# Autodesk Inventor assembly: LinearLift12in
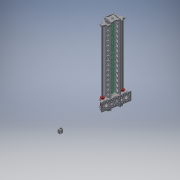
[picture p0: Inventor's stored thumbnail of the model, 180x180]
Saved by Autodesk Inventor 2018 (Build 220112000, 112)
## iProperties
Created: 2017-11-27
Part Number: LinearLift12in
Document SubType Name: Assembly
Designer: ball
Author: ball
## Documents named in this file (12)
- C:\FTC\FTC8863CAD\2017Robot\LinearLift12in.iam
- C:\FTC\FTC8863CAD\Actobotics\585 parts\585456.ipt
- C:\FTC\FTC8863CAD\Actobotics\585 parts\585634.ipt
- C:\FTC\FTC8863CAD\Actobotics\634 parts\634314.ipt
- C:\FTC\FTC8863CAD\Actobotics\535 parts\535094 assembly.ipt
- C:\FTC\FTC8863CAD\Actobotics\634 parts\634050.ipt
- C:\FTC\FTC8863CAD\Actobotics\545 parts\545314.ipt
- C:\FTC\FTC8863CAD\Actobotics\585 parts\585546.ipt
- C:\FTC\FTC8863CAD\Actobotics\535 parts\535226.ipt
- C:\FTC\FTC8863CAD\Actobotics\585 parts\585640.ipt
- C:\FTC\FTC8863CAD\Actobotics\585 parts\585722.ipt
- C:\FTC\FTC8863CAD\Actobotics\525 parts\625052 assembly.ipt
## Components (19 placed, 11 different names)
1. 585456:1 — Mate:1, Mate:2, Mate:3, Mate:7, Mate:8, Mate:9, Mate:10, Mate:14, Mate:15, Mate:16, Mate:17, Mate:38, Mate:39, Mate:40, Mate:41
2. 585634:1 — Mate:7, Mate:37, Mate:38, Mate:39
3. 585634:2 — Mate:1, Mate:2, Mate:3, Mate:4, Flush:1
4. 585634:3 — Mate:8, Mate:9, Mate:10, Mate:11, Flush:2
5. 585634:4 — Mate:14, Mate:40, Mate:41
6. 634314:1 — Mate:4, Flush:1, Mate:19
7. 634314:2 — Mate:11, Flush:2, Mate:20
8. 535094 assembly:1 — Mate:15, Mate:16, Mate:17, Flush:3, Mate:35
9. 634050:1 — Flush:3, Cylindrical:1, Mate:35
10. 545314:1 — Cylindrical:1, Mate:18, Flush:4
11. 585546:1 — Mate:18, Flush:4, Flush:8, Mate:36
12. 535226:1 — Mate:19, Flush:6, Mate:21, Flush:9, Mate:37
13. 535226:2 — Mate:20, Flush:6, Mate:22
14. 585640:2 — Mate:21, Mate:33, Flush:9
15. 585640:3 — Mate:22, Flush:8, Mate:31, Mate:32, Mate:34
16. 585722:1 — Mate:25, Mate:26, Mate:27, Mate:28, Mate:29, Mate:30, Mate:31, Mate:32, Mate:33, Mate:34, Mate:36
17. 585640:4 — Mate:25, Mate:26, Mate:27
18. 585640:5 — Mate:28, Mate:29, Mate:30
19. 625052 assembly:1
## Relationships (43: Mate 35, Flush 7, CylindricalJoint 1)
- Mate:1: 585456:1 ↔ 585634:2
- Mate:2: 585456:1 ↔ 585634:2
- Mate:3: 585456:1 ↔ 585634:2
- Mate:4: 585634:2 ↔ 634314:1
- Flush:1: 585634:2 ↔ 634314:1
- Mate:7: 585456:1 ↔ 585634:1
- Mate:8: 585456:1 ↔ 585634:3
- Mate:9: 585456:1 ↔ 585634:3
- Mate:10: 585456:1 ↔ 585634:3
- Mate:11: 585634:3 ↔ 634314:2
- Flush:2: 585634:3 ↔ 634314:2
- Mate:14: 585456:1 ↔ 585634:4
- Mate:15: 585456:1 ↔ 535094 assembly:1
- Mate:16: 585456:1 ↔ 535094 assembly:1
- Mate:17: 585456:1 ↔ 535094 assembly:1
- Flush:3: 535094 assembly:1 ↔ 634050:1
- Cylindrical:1: 634050:1 ↔ 545314:1
- Mate:18: 545314:1 ↔ 585546:1
- Flush:4 (-3.175 mm): 545314:1 ↔ 585546:1
- Mate:19: 634314:1 ↔ 535226:1
- Mate:20: 634314:2 ↔ 535226:2
- Flush:6: 535226:1 ↔ 535226:2
- Mate:21: 535226:1 ↔ 585640:2
- Mate:22: 535226:2 ↔ 585640:3
- Flush:8: 585546:1 ↔ 585640:3
- Mate:25: 585722:1 ↔ 585640:4
- Mate:26: 585722:1 ↔ 585640:4
- Mate:27: 585722:1 ↔ 585640:4
- Mate:28: 585722:1 ↔ 585640:5
- Mate:29: 585722:1 ↔ 585640:5
- Mate:30: 585722:1 ↔ 585640:5
- Mate:31: 585640:3 ↔ 585722:1
- Mate:32: 585640:3 ↔ 585722:1
- Mate:33: 585640:2 ↔ 585722:1
- Mate:34: 585640:3 ↔ 585722:1
- Mate:35: 535094 assembly:1 ↔ 634050:1
- Mate:36: 585546:1 ↔ 585722:1
- Flush:9 (5.7912 mm): 535226:1 ↔ 585640:2
- Mate:37: 585634:1 ↔ 535226:1
- Mate:38: 585456:1 ↔ 585634:1
- Mate:39: 585456:1 ↔ 585634:1
- Mate:40: 585456:1 ↔ 585634:4
- Mate:41: 585456:1 ↔ 585634:4
